# Autodesk Inventor assembly: leg_ass_1
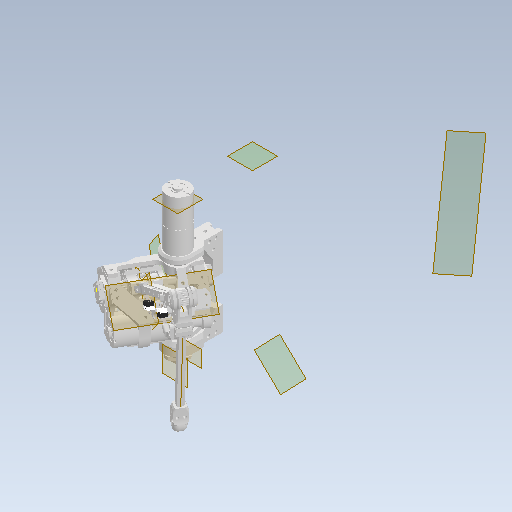
[picture p0: Inventor's stored thumbnail of the model, 512x512]
Saved by Autodesk Inventor 2020 (Build 240168000, 168)
## iProperties
Created: 2019-05-04
Part Number: leg_ass_1
Document SubType Name: Assembly
Designer: psrob
Author: psrob
## Documents named in this file (13)
- E:\projects-2\project dog gen2\hardware\leg_ass_1.iam
- E:\projects-2\project dog gen2\hardware\leg_bone_2.iam
- E:\projects-2\project dog gen2\hardware\leg_bone_1.iam
- E:\projects-2\project dog gen2\hardware\2GT_wheel.ipt
- E:\projects-2\project dog gen2\hardware\bearing_6_10_3.ipt
- E:\projects-2\project dog gen2\hardware\leg_motor_moudle.iam
- E:\projects-2\project dog gen2\hardware\dog_bone_1.ipt
- E:\projects-2\project dog gen2\hardware\motor_2.ipt
- E:\projects-2\project dog gen2\hardware\dog_bone_3.ipt
- E:\projects-2\project dog gen2\hardware\encoder_ass.iam
- E:\projects-2\project dog gen2\hardware\switch_holder_1.ipt
- E:\projects-2\project dog gen2\hardware\ultra-subminiature-basic-switch-d2f-1.snapshot.2\D2F-01L.ipt
- E:\projects-2\project dog gen2\hardware\switch_holder_3.ipt
## Components (14 placed, 12 different names)
1. leg_bone_2:1 [sub-assembly] — Insert:1, Insert:3, Insert:4, Insert:5, Insert:6, Angle:5, Angle:6
2. leg_bone_1:1 [sub-assembly] — Insert:1, Angle:5
3. 2GT_wheel:1 — Insert:5
4. bearing_6_10_3:1 — Insert:3
5. bearing_6_10_3:2 — Insert:4
6. leg_motor_moudle:1 [sub-assembly] — Insert:6, Insert:8, Insert:9, Flush:3, Angle:4, Tangent:2, Angle:6, Angle:7, Flush:6, Insert:15, Insert:16
7. dog_bone_1:1 — Insert:9, Flush:1, Angle:1, Insert:10, Insert:11
8. motor_2:1 — Insert:8, Mate:1, Tangent:1, Flush:2
9. dog_bone_3:1 — Flush:1, Mate:1, Angle:1, Tangent:1, Angle:7, Mate:2, Flush:4, Flush:5
10. encoder_ass:1 [sub-assembly] — Insert:10, Insert:11
11. switch_holder_1:1 — Flush:3, Angle:4, Insert:13, Insert:14, Tangent:2
12. D2F-01L:1 — Insert:13, Insert:14
13. D2F-01L:2 — Mate:2, Flush:4, Flush:5
14. switch_holder_3:1 — Flush:6, Insert:15, Insert:16
## Relationships (28: Insert 13, Flush 6, Angle 5, Mate 2, Tangent 2)
- Insert:1: leg_bone_2:1 ↔ leg_bone_1:1
- Insert:3: leg_bone_2:1 ↔ bearing_6_10_3:1
- Insert:4: leg_bone_2:1 ↔ bearing_6_10_3:2
- Insert:5 (0.5 mm): leg_bone_2:1 ↔ 2GT_wheel:1
- Insert:6 (0.5 mm): leg_bone_2:1 ↔ leg_motor_moudle:1
- Insert:8 (-12 mm): leg_motor_moudle:1 ↔ motor_2:1
- Insert:9: leg_motor_moudle:1 ↔ dog_bone_1:1
- Flush:1: dog_bone_1:1 ↔ dog_bone_3:1
- Mate:1: motor_2:1 ↔ dog_bone_3:1
- Angle:1 (0 deg): dog_bone_1:1 ↔ dog_bone_3:1
- Tangent:1: motor_2:1 ↔ dog_bone_3:1
- Insert:10: dog_bone_1:1 ↔ encoder_ass:1
- Insert:11: dog_bone_1:1 ↔ encoder_ass:1
- Flush:2 (-10 mm): motor_2:1
- Flush:3: leg_motor_moudle:1 ↔ switch_holder_1:1
- Angle:4 (0 deg): leg_motor_moudle:1 ↔ switch_holder_1:1
- Insert:13: switch_holder_1:1 ↔ D2F-01L:1
- Insert:14: switch_holder_1:1 ↔ D2F-01L:1
- Tangent:2: leg_motor_moudle:1 ↔ switch_holder_1:1
- Angle:5 (235 deg): leg_bone_2:1 ↔ leg_bone_1:1
- Angle:6 (120 deg): leg_bone_2:1 ↔ leg_motor_moudle:1
- Angle:7 (-60 deg): leg_motor_moudle:1 ↔ dog_bone_3:1
- Mate:2 (15 mm): dog_bone_3:1 ↔ D2F-01L:2
- Flush:4 (-2 mm): dog_bone_3:1 ↔ D2F-01L:2
- Flush:5 (5 mm): dog_bone_3:1 ↔ D2F-01L:2
- Flush:6: leg_motor_moudle:1 ↔ switch_holder_3:1
- Insert:15: leg_motor_moudle:1 ↔ switch_holder_3:1
- Insert:16: leg_motor_moudle:1 ↔ switch_holder_3:1
